# Autodesk Inventor assembly: 0913-DX(R,D-129)(F,D-166-1)
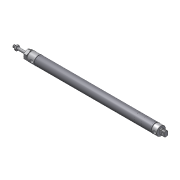
[picture p0: Inventor's stored thumbnail of the model, 180x180]
Saved by Autodesk Inventor 2012 (Build 160160000, 160)
## iProperties
Category: PARTsolutions
Created: 2013-01-19
Part Number: 0913-DX(R,D-129)(F,D-166-1)
Catalog Web Link: www.cadenas.de
Description: Original Line Standard Air Cylinders -
Document SubType Name: Assembly
Designer: PARTsolutions
Mass: 201.797 g
Surface Area: 894.204 cm^2
Volume: 82.7162 cm^3
Density: 2.43964 g/cm^3
NB: 0913-DX(R,D-129)(F,D-166-1)
NN: Original Line Standard Air Cylinders
NBSYN: $PNC.
LINA: 0913-DX
PSOL_MULTISOLIDPART: 0.0
PN: 0913-DX
PNC: 0913-DX(R,D-129)(F,D-166-1)
PNA: (D-129)(D-166-1)
DASH: -
BORE1: 1.06250000
BORE: 1 1/16" (09)
BOREPN: 09
STROKE: 13.000
STROKEALG: [0.011:50/0.001]
STROKE1: 13.000
ACTING: D
ACTINGALG: '' , 'Single Acting (SA)' , 'R' , 'Reverse Single Acting (SA)' , 'D' , 'Double Acting (SA)'
ACTINGPN: D
MNT: X
MNTALG: '' , 'Front Nose Mounting (SA)' , 'P' , 'Rear Pivot Mounting (SA)' , 'X' , 'Universal Pivot Mounting or Double End Mounting (SA)' , 'BF' , 'Front Block Mounting (SA)' , 'BR' , 'Rear Block Mounting for Vertical Positioning (SA)' , 'BFT' , 'Front Block Trunnion Mounting (SA)' , 'BRT' , 'Rear Block Trunnion Mounting (SA)'
MNTPN: X
DERALG: '' , 'Standard Single End Rod' , 'DE' , 'With Double End Rod' , 'DEH' , 'With Double End Hollow Rod'
NRALG: '' , 'N/A'
BMALG: '' , 'N/A'
COALG: '' , 'N/A'
OOALG: '', 'N/A'
VO: Z
VOALG: 'Z' , 'N/A'
MALG: '', 'Without Magnet', 'M', 'With Magnet'
EEL: 0.000
EEMAX: 37.0000
EEALG: '', 'Without Extra Extension', 'EE', 'With Extra Extension'
EELALG: 0
EEPN1: 0.000
KALG: '', 'Standard' , 'K' , 'Ports Rotated 90deg K'
QALG: '' , 'N/A'
YALG: '' , 'Without Pivot Bushing' , 'Y' , 'With Pivot Bushing'
FALG: '', 'Non-Coated (Standard)', 'F', 'Molycoated'
TALG: '' , 'Standard -20° to 200°F (-29° to 95°C)' , 'N' , 'Low Temperature' , 'V' , 'High Temperature'
BALG: '', 'W/out Bumpers' , 'B' , 'W/ Bumpers'
HALG: '', 'N/A'
SERALG: '' , 'Without Spring Extend/Return' , 'JS' , 'With Spring Return' , 'JR' , 'With Spring Extend'
SRALG: '' , 'Standard Stainless Steel'
SRCON: 0
WALG: '' , 'Without Wiper' , 'W' , 'With Wiper'
EALG: '' , 'Standard Seals/Lube' , 'E' , 'Non-Lube Seals/Lube'
HLALG: '' , 'Without Low Pressure Hydraulic' , 'HL' , 'With Low Pressure Hydraulic'
STALG: '' , 'N/A'
STPT1ALG: '' , 'N/A'
STPT2ALG: '' , 'N/A'
STPT3ALG: '' , 'N/A'
STPT4ALG: '' , 'N/A'
MB: R,D-129
MBALG: '' , 'Without Mounting Bracket' , 'F,D-129' , 'D-129 (front)'  , 'R,D-129' , 'D-129 (rear)' , '2x,D-129' , 'D-129 (front & rear)'
MBPN: (R,D-129)
MBPNALL: D-129
MBPNALLREAR: D-129
PBALG: '' , 'N/A'
PBPNALL: D-13498-A
PRC: F,D-166-1
PRCALG: '' , 'W/out Pivot Rod Clevis' , 'F,D-166-1' , 'D-166-1 (front)'
PRCPN: (F,D-166-1)
PRCPNALL: D-166-1
TBALG: '' , 'N/A'
MNALG: '' , 'N/A'
TLEN: 14.3185
FRAC: 184.8400
RGDACCON: R
RHCON: P
RHCON1: P
RHCONON: 1
FNUTCON: 1
RNUTCON: 1
FNUTPN: D-9
RNUTPN: D-9
FNUTTRANS: 0.0000
RNUTTRANS: 0.0000
VHOLECON: 0
A1: 1.6250
A1N: 1.0000
A1P: 1.6250
A1B: 1.8750
A4: 0.2525
A4N: 0.3750
A4P: 0.2525
A5: 0.0300
A1H: 1.500
A1NH: 0.6250
A1PH: 1.5000
A1BH: 1.1250
A1SH: 1.1250
A2H: 0.2500
A2NH: 0.2500
LENGTH: 3.8400
LENGTH1: 3.8400
LENGTH2: 4.1000
MUL: 13.0000
MUL11: 13.0000
MUL22: 33.280
MUL33: 20.2800
MUL2: 13.0000
MUL211: 13.0000
MUL222: 2.5600
MUL233: 1.5600
SSS: 26.0000
RGLEN: 1.4025
RHLEN: 0.9990
SSS1: 14.0000
A13: 1.2190
DIF: 0.1200
G5: 0.7180
ON: 0
SSADD: 0.0000
BADD: 0.0000
MADD: 0.0000
NVADD: 0.0000
TRACKL: 14.0285
TRACKCON: D-78527
TRIMCON: 0
TRIMCON1: 0
FSPACE: 1.0801
SPACE: 0.2580
TEXT: 0.4516
S1: 1.2500
D1: 1.1410
D1N: 1.1130
D1B: 1.1130
D1P: 1.1410
FA: 0.940
RA: 0.9400
PPATH: standard_air_cylinder_asmtpl.prj
MATALGHTML: <b>Standard Original Line:</b><dl><dt>Rod:</dt><dd>- Stainless Steel</dd><dd>&nbsp;&nbsp;(5/16 ? 9/16 Bores)</dd><dd>- High Strength Carbon Steel</dd><dd>&nbsp;&nbsp;(3/4 ? 3 Bore)</dd><dd>- Stainless Steel</dd><dd>&nbsp;&nbsp;(?X? style DXP/DX/DXDE?)</dd><dt>Bearings:</dt><dd>- Sintered Bronze</dd><dt>Body:</dt><dd>- 304 Stainless Steel</dd><dt>End Caps:</dt><dd>- Aluminum</dd><dt>Seals:</dt><dd>- Buna N</dd></dl>
ASSCFGPRA: 09DX
MBPNA: (D-129)
PRCPNA: (D-166-1)
ASSOPTACC: STPT4
A: 16.84
HADD: 0.0000
WFL: 0.125
QADD: 0.000
QADD1: 0.250
TEST: 13.0000
STDNUTF: 1
STDNUTR: 1
KT: DUMMY
CreationOption_UseAsmMates: false
SUPPLIER: Bimba
ARTICLENO: 0913-DX(R,D-129)(F,D-166-1)
BOMINFO: 0913-DX
CREATOR: CADENAS GmbH
PSOL_IDENT_0: {\\10.0.0.242\data_v9\23d-libs\bimba\bimba\bimba_imperial\bimba_full_line\original_line_cylinders\st
PSOL_IDENT_1: andard_air_cylinders\standard_air_cylinder_asmtab.prj},325 {VTYP=3D},{STYP=ASSTAB},{NB=0913-DX(R,D-1
PSOL_IDENT_2: 29)(F,D-166-1)},{LINA=0913-DX},{NN=Original Line Standard Air Cylinders},{DATE=06.09.2012 11:26:56},
PSOL_IDENT_3: {GEOMDATE=06.09.2012},{VERSION=},{LINEID=10},{LINESUBID=-1},{WBVAR=STROKE,ACTING,MNT,DER,NR,BM,CO,OO
PSOL_IDENT_4: ,VO,M,EE,EEL,K,Q,Y,G,T,B,H,SER,SR,NT,W,HL,STPT1,STPT2,STPT3,STPT4,MB,PB,PRC,TB,MN}  {NB=0913-DX(R,D-
PSOL_IDENT_5: 129)(F,D-166-1)},{LINA=0913-DX},{KT=DUMMY},{PN=0913-DX},{PNC=0913-DX(R,D-129)(F,D-166-1)},{PNA=(D-12
PSOL_IDENT_6: 9)(D-166-1)},{DASH=-},{BORE1=1.06250000},{BORE=1 1/16\" (09)},{BOREPN=09},{STROKE=13.000},{STROKEALG
PSOL_IDENT_7: =[0.011:50/0.001]},{STROKE1=13.000},{ACTING=D},{ACTINGALG= '' , 'Single Acting (SA)' , 'R' , 'Revers
PSOL_IDENT_8: e Single Acting (SA)' , 'D' , 'Double Acting (SA)' },{ACTINGPN=D},{MNT=X},{MNTALG= '' , 'Front Nose
PSOL_IDENT_9: Mounting (SA)' , 'P' , 'Rear Pivot Mounting (SA)' , 'X' , 'Universal Pivot Mounting or Double End Mo
PSOL_IDENT_10: unting (SA)' , 'BF' , 'Front Block Mounting (SA)' , 'BR' , 'Rear Block Mounting for Vertical Positio
PSOL_IDENT_11: ning (SA)' , 'BFT' , 'Front Block Trunnion Mounting (SA)' , 'BRT' , 'Rear Block Trunnion Mounting (S
PSOL_IDENT_12: A)' },{TYPE=},{MNTPN=X},{DER=},{DERALG= '' , 'Standard Single End Rod' , 'DE' , 'With Double End Rod
PSOL_IDENT_13: ' , 'DEH' , 'With Double End Hollow Rod' },{NR=},{NRALG= '' , 'N/A' },{NRPN=},{BM=},{BMALG= '' , 'N/
PSOL_IDENT_14: A' },{BMPN=},{CO=},{COALG= '' , 'N/A' },{OO=},{OOALG= '', 'N/A' },{OOPN=},{VO=Z},{VOALG= 'Z' , 'N/A'
PSOL_IDENT_15: },{VOPN=},{OOVOPN=},{M=},{MALG= '', 'Without Magnet', 'M', 'With Magnet' },{EE=},{EEL=0.000},{EEMAX
PSOL_IDENT_16: =37.0000},{EEALG= '', 'Without Extra Extension', 'EE', 'With Extra Extension' },{EELALG=0},{EEPN=},{
PSOL_IDENT_17: EEPN1=0.000},{K=},{KALG= '', 'Standard' , 'K' , 'Ports Rotated 90deg K' },{KPN=},{Q=},{QALG= '' , 'N
PSOL_IDENT_18: /A' },{QPN=},{Y=},{YALG= '' , 'Without Pivot Bushing' , 'Y' , 'With Pivot Bushing' },{YPN=},{YCON=},
PSOL_IDENT_19: {F=},{FALG= '', 'Non-Coated (Standard)', 'F', 'Molycoated' },{FPN=},{G=},{GPN=},{GPN99=},{T=},{TALG=
PSOL_IDENT_20: '' , 'Standard -20° to 200°F (-29° to 95°C)' , 'N' , 'Low Temperature' , 'V' , 'High Temperature' }
PSOL_IDENT_21: ,{NPN=},{VPN=},{B=},{BALG= '', 'W/out Bumpers' , 'B' , 'W/ Bumpers' },{BPN=},{H=},{HALG= '', 'N/A' }
PSOL_IDENT_22: ,{HPN=},{SER=},{SERALG= '' , 'Without Spring Extend/Return' , 'JS' , 'With Spring Return' , 'JR' , '
PSOL_IDENT_23: With Spring Extend' },{SR=},{SRALG= '' , 'Standard Stainless Steel' },{SRPN=},{SRCON=0},{NT=},{NTPN=
PSOL_IDENT_24: },{W=},{WALG= '' , 'Without Wiper' , 'W' , 'With Wiper' },{WPN=},{E=},{EALG= '' , 'Standard Seals/Lu
PSOL_IDENT_25: be' , 'E' , 'Non-Lube Seals/Lube' },{EPN=},{HL=},{HLALG= '' , 'Without Low Pressure Hydraulic' , 'HL
PSOL_IDENT_26: ' , 'With Low Pressure Hydraulic' },{ST=},{STALG= '' , 'N/A' },{STPT1=},{STPT1ALG= '' , 'N/A' },{STP
PSOL_IDENT_27: T2=},{STPT2ALG= '' , 'N/A' },{STPT3=},{STPT3ALG= '' , 'N/A' },{STPT4=},{STPT4ALG= '' , 'N/A' },{STPN
PSOL_IDENT_28: =},{MB=R,D-129},{MBALG= '' , 'Without Mounting Bracket' , 'F,D-129' , 'D-129 (front)'  , 'R,D-129' ,
PSOL_IDENT_29: 'D-129 (rear)' , '2x,D-129' , 'D-129 (front & rear)'},{MBPN=(R,D-129)},{MBPNALL=D-129},{MBPNALLREAR
PSOL_IDENT_30: =D-129},{PB=},{PBALG= '' , 'N/A' },{PBPN=},{PBPNALL=D-13498-A},{PRC=F,D-166-1},{PRCALG= '' , 'W/out
PSOL_IDENT_31: Pivot Rod Clevis' , 'F,D-166-1' , 'D-166-1 (front)' },{PRCPN=(F,D-166-1)},{PRCPNALL=D-166-1},{TB=},{
PSOL_IDENT_32: TBALG= '' , 'N/A' },{TBPN=},{TBPNALL=},{MN=},{MNALG= '' , 'N/A' },{MNPN=},{MNCONF=},{MNCONR=},{TLEN=
PSOL_IDENT_33: 14.3185},{FRAC=184.8400},{RGCON=},{RGDACCON=R},{RHCON=P},{RHCON1=P},{RHCONON=1},{RHACCON=},{FNUTCON=
PSOL_IDENT_34: 1},{RNUTCON=1},{FNUTPN=D-9},{RNUTPN=D-9},{FNUTTRANS=0.0000},{RNUTTRANS=0.0000},{VHOLECON=0},{A1=1.62
PSOL_IDENT_35: 50},{A1N=1.0000},{A1P=1.6250},{A1B=1.8750},{A4=0.2525},{A4N=0.3750},{A4P=0.2525},{A5=0.0300},{A1H=1.
PSOL_IDENT_36: 5},{A1NH=0.6250},{A1PH=1.5000},{A1BH=1.1250},{A1SH=1.1250},{A2H=0.2500},{A2NH=0.2500},{LENGTH=3.8400
PSOL_IDENT_37: },{LENGTH1=3.8400},{LENGTH2=4.1000},{MUL=13.0000},{MUL11=13.0000},{MUL22=33.28},{MUL33=20.2800},{MUL
PSOL_IDENT_38: 2=13.0000},{MUL211=13.0000},{MUL222=2.5600},{MUL233=1.5600},{SSS=26.0000},{RGLEN=1.4025},{RHLEN=0.99
PSOL_IDENT_39: 90},{SSS1=14.0000},{A13=1.2190},{DIF=0.1200},{G5=0.7180},{ON=0},{SSADD=0.0000},{BADD=0.0000},{MADD=0
PSOL_IDENT_40: .0000},{NVADD=0.0000},{TRACKL=14.0285},{TRACKCON=D-78527},{TRIMCON=0},{TRIMCON1=0},{PINCON=},{FSPACE
PSOL_IDENT_41: =1.0801},{SPACE=0.2580},{TEXT=0.4516},{S1=1.2500},{D1=1.1410},{D1N=1.1130},{D1B=1.1130},{D1P=1.1410}
PSOL_IDENT_42: ,{FA=0.940},{RA=0.9400},{PPATH=standard_air_cylinder_asmtpl.prj},{MATALGHTML=<b>Standard Original Li
PSOL_IDENT_43: ne:</b><dl><dt>Rod:</dt><dd>- Stainless Steel</dd><dd>&nbsp;&nbsp;(5/16 ? 9/16 Bores)</dd><dd>- High
PSOL_IDENT_44: Strength Carbon Steel</dd><dd>&nbsp;&nbsp;(3/4 ? 3 Bore)</dd><dd>- Stainless Steel</dd><dd>&nbsp;&n
PSOL_IDENT_45: bsp;(?X? style DXP/DX/DXDE?)</dd><dt>Bearings:</dt><dd>- Sintered Bronze</dd><dt>Body:</dt><dd>- 304
PSOL_IDENT_46: Stainless Steel</dd><dt>End Caps:</dt><dd>- Aluminum</dd><dt>Seals:</dt><dd>- Buna N</dd></dl>},{AS
PSOL_IDENT_47: SCFGPRA=09DX},{MBPNA=(D-129)},{MNPNA=},{PRCPNA=(D-166-1)},{ASSOPTACC=STPT4},{A=16.84},{HADD=0.0000},
PSOL_IDENT_48: {WFL=0.125},{QADD=0.000},{QADD1=0.250},{TEST=13.0000},{MNTB=},{STDNUTF=1},{STDNUTR=1}
Title: 0913-DX
Author: Cadenas PARTsolutions
## Documents named in this file (8)
- Z:\UserData\Documents\Inventor\team1885frc\Pneumatics\0913-DX_13inStrokex10625Bore\0913_DX_R_D_129__F_D_166_1_.iam
- Z:\UserData\Documents\Inventor\team1885frc\Pneumatics\0913-DX_13inStrokex10625Bore\09R000_rod_guide.ipt
- Z:\UserData\Documents\Inventor\team1885frc\Pneumatics\0913-DX_13inStrokex10625Bore\0913_DX0_rod.ipt
- Z:\UserData\Documents\Inventor\team1885frc\Pneumatics\0913-DX_13inStrokex10625Bore\D_166_1_dummy.ipt
- Z:\UserData\Documents\Inventor\team1885frc\Pneumatics\0913-DX_13inStrokex10625Bore\D_746.ipt
- Z:\UserData\Documents\Inventor\team1885frc\Pneumatics\0913-DX_13inStrokex10625Bore\09R_14_31350.ipt
- Z:\UserData\Documents\Inventor\team1885frc\Pneumatics\0913-DX_13inStrokex10625Bore\09P0010_rear_head.ipt
- Z:\UserData\Documents\Inventor\team1885frc\Pneumatics\0913-DX_13inStrokex10625Bore\D_9.ipt
## Components (7 placed, 7 different names)
1. 09R000_rod_guide:1 — Mate:1
2. D-166-1-dummy:1
3. 09R-14.31350:1
4. 09P0010_rear_head:1 — Mate:2
5. D-9:2
6. D-746:1 — Mate:3, Mate:4
7. 0913-DX0_rod:1 — Mate:1, Mate:2, Mate:3, Mate:4
## Relationships (4: Mate 4)
- Mate:1: 09R000_rod_guide:1 ↔ 0913-DX0_rod:1
- Mate:2: 09P0010_rear_head:1 ↔ 0913-DX0_rod:1
- Mate:3: D-746:1 ↔ 0913-DX0_rod:1
- Mate:4: D-746:1 ↔ 0913-DX0_rod:1
